# Autodesk Inventor assembly: gp2_block
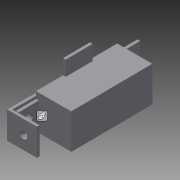
[picture p0: Inventor's stored thumbnail of the model, 180x180]
Saved by Autodesk Inventor 2015 (Build 190159000, 159)
## iProperties
Created: 2015-10-17
Part Number: gp2_block
Document SubType Name: Assembly
Designer: astralien3000
Author: astralien3000
## Documents named in this file (3)
- C:\Users\astralien3000\Desktop\ceres\meca\v2016\gp2_block.iam
- C:\Users\astralien3000\Desktop\ceres\meca\lib\struct\equerre.ipt
- C:\Users\astralien3000\Desktop\ceres\meca\lib\sensor\gp2.ipt
## Components (2 placed, 2 different names)
1. equerre:1 — Placage:1, Placage:2, Placage:3, Placage:4, Placage:5
2. gp2:1 — Placage:4, Placage:5
## Relationships (5: Mate 5)
- Placage:1 [Mate]: equerre:1
- Placage:2 [Mate]: equerre:1
- Placage:3 [Mate]: equerre:1
- Placage:4 [Mate]: equerre:1 ↔ gp2:1
- Placage:5 [Mate]: equerre:1 ↔ gp2:1
